# Autodesk Inventor assembly: Test mechanum wheel drive train
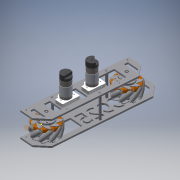
[picture p0: Inventor's stored thumbnail of the model, 180x180]
Saved by Autodesk Inventor 2017 (Build 210142000, 142)
## iProperties
Created: 2017-08-02
Part Number: Test mechanum wheel drive train
Document SubType Name: Assembly
Designer: User
Author: User
## Documents named in this file (7)
- C:\Robotics\CAD\2016-17_CAD\Test mechanum wheel drive train.iam
- C:\Robotics\CAD\2016-17_CAD\DriveTrain\DrainTrainPlate2.0LeftOutside.iam
- C:\Robotics\CAD\2016-17_CAD\DriveTrain\wheel sub assembly mechanum wheels .iam
- C:\Robotics\CAD\2016-17_CAD\DriveTrain\DriveTrainPlate2.0LeftInside.ipt
- C:\Robotics\CAD\2016-17_CAD\DriveTrain\motor sub assembley.iam
- C:\Robotics\CAD\COTSParts\Tetrix\tetrix-motor-mounts-1.snapshot.1\Tetrex 2pc motor mount.ipt
- C:\Robotics\CAD\2016-17_CAD\DriveTrain\drive train standoff.0002.ipt
## Components (11 placed, 6 different names)
1. DrainTrainPlate2.0LeftOutside:1 [sub-assembly] — Mate:3, Mate:4, Mate:5, Mate:8
2. wheel sub assembly mechanum wheels :1 [sub-assembly] — Mate:6, Mate:7, Mate:8, Flush:1, Flush:2
3. wheel sub assembly mechanum wheels :2 [sub-assembly] — Mate:1, Mate:2, Mate:3, Mate:4, Mate:5, Flush:3
4. DriveTrainPlate2.0LeftInside:1 — Mate:1, Mate:2, Mate:6, Mate:7, Mate:9, Insert:1, Mate:11, Insert:2, Mate:13, Mate:14, Mate:15, Mate:16, Mate:17, Mate:18
5. motor sub assembley:1 [sub-assembly] — Flush:1, Mate:9, Flush:2, Mate:10
6. motor sub assembley:2 [sub-assembly] — Mate:11, Flush:3, Mate:12
7. Tetrex 2pc motor mount:1 — Mate:10, Insert:1
8. Tetrex 2pc motor mount:2 — Mate:12, Insert:2
9. drive train standoff.0002:1 — Mate:17, Mate:18
10. drive train standoff.0002:2 — Mate:13, Mate:14
11. drive train standoff.0002:3 — Mate:15, Mate:16
## Relationships (23: Mate 18, Flush 3, Insert 2)
- Mate:1 (6.35 mm): wheel sub assembly mechanum wheels :2 ↔ DriveTrainPlate2.0LeftInside:1
- Mate:2: wheel sub assembly mechanum wheels :2 ↔ DriveTrainPlate2.0LeftInside:1
- Mate:3: DrainTrainPlate2.0LeftOutside:1 ↔ wheel sub assembly mechanum wheels :2
- Mate:4: DrainTrainPlate2.0LeftOutside:1 ↔ wheel sub assembly mechanum wheels :2
- Mate:5: DrainTrainPlate2.0LeftOutside:1 ↔ wheel sub assembly mechanum wheels :2
- Mate:6 (6.35 mm): wheel sub assembly mechanum wheels :1 ↔ DriveTrainPlate2.0LeftInside:1
- Mate:7: wheel sub assembly mechanum wheels :1 ↔ DriveTrainPlate2.0LeftInside:1
- Mate:8: DrainTrainPlate2.0LeftOutside:1 ↔ wheel sub assembly mechanum wheels :1
- Flush:1: wheel sub assembly mechanum wheels :1 ↔ motor sub assembley:1
- Mate:9: DriveTrainPlate2.0LeftInside:1 ↔ motor sub assembley:1
- Flush:2: wheel sub assembly mechanum wheels :1 ↔ motor sub assembley:1
- Mate:10: motor sub assembley:1 ↔ Tetrex 2pc motor mount:1
- Insert:1: DriveTrainPlate2.0LeftInside:1 ↔ Tetrex 2pc motor mount:1
- Mate:11: DriveTrainPlate2.0LeftInside:1 ↔ motor sub assembley:2
- Flush:3: wheel sub assembly mechanum wheels :2 ↔ motor sub assembley:2
- Mate:12: motor sub assembley:2 ↔ Tetrex 2pc motor mount:2
- Insert:2: DriveTrainPlate2.0LeftInside:1 ↔ Tetrex 2pc motor mount:2
- Mate:13: DriveTrainPlate2.0LeftInside:1 ↔ drive train standoff.0002:2
- Mate:14: DriveTrainPlate2.0LeftInside:1 ↔ drive train standoff.0002:2
- Mate:15: DriveTrainPlate2.0LeftInside:1 ↔ drive train standoff.0002:3
- Mate:16: DriveTrainPlate2.0LeftInside:1 ↔ drive train standoff.0002:3
- Mate:17: DriveTrainPlate2.0LeftInside:1 ↔ drive train standoff.0002:1
- Mate:18: DriveTrainPlate2.0LeftInside:1 ↔ drive train standoff.0002:1
